# Autodesk Inventor assembly: led bar assembly
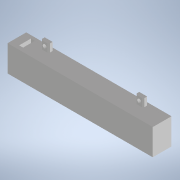
[picture p0: Inventor's stored thumbnail of the model, 180x180]
Saved by Autodesk Inventor 2022 (Build 260153000, 153)
## iProperties
Created: 2022-04-16
Part Number: led bar assembly
Document SubType Name: Assembly
Designer: a-dubs
Author: a-dubs
## Documents named in this file (5)
- W:\My Drive\Coding and Projects\smart home\smart-deadbolt\3D Modelling\led bar assembly.iam
- W:\My Drive\Coding and Projects\smart home\smart-deadbolt\3D Modelling\10x led strip holder .ipt
- W:\My Drive\Coding and Projects\smart home\smart-deadbolt\3D Modelling\10x led strip holder top cover.ipt
- W:\My Drive\Coding and Projects\smart home\smart-deadbolt\3D Modelling\10x led strip grid divider opaque.ipt
- W:\My Drive\Coding and Projects\smart home\smart-deadbolt\3D Modelling\1x led strip diffuser.ipt
## Components (13 placed, 4 different names)
1. 10x led strip holder :1 — Mate:7, Mate:8
2. 10x led strip holder top cover:1 — Mate:4, Mate:5, Mate:6, Mate:7, Mate:8
3. 10x led strip grid divider opaque:1 — Mate:1, Mate:2, Mate:3
4. 1x led strip diffuser:1 — Mate:1, Mate:2, Mate:3, Mate:4, Mate:5, Mate:6
5. 1x led strip diffuser:2
6. 1x led strip diffuser:3
7. 1x led strip diffuser:4
8. 1x led strip diffuser:5
9. 1x led strip diffuser:6
10. 1x led strip diffuser:7
11. 1x led strip diffuser:8
12. 1x led strip diffuser:9
13. 1x led strip diffuser:10
## Component patterns: (10 elements, first: 1x led strip diffuser:1)
## Relationships (8: Mate 8)
- Mate:1: 10x led strip grid divider opaque:1 ↔ 1x led strip diffuser:1
- Mate:2: 10x led strip grid divider opaque:1 ↔ 1x led strip diffuser:1
- Mate:3: 10x led strip grid divider opaque:1 ↔ 1x led strip diffuser:1
- Mate:4: 10x led strip holder top cover:1 ↔ 1x led strip diffuser:1
- Mate:5: 10x led strip holder top cover:1 ↔ 1x led strip diffuser:1
- Mate:6: 10x led strip holder top cover:1 ↔ 1x led strip diffuser:1
- Mate:7: 10x led strip holder :1 ↔ 10x led strip holder top cover:1
- Mate:8: 10x led strip holder :1 ↔ 10x led strip holder top cover:1
